# Autodesk Inventor assembly: 3段目
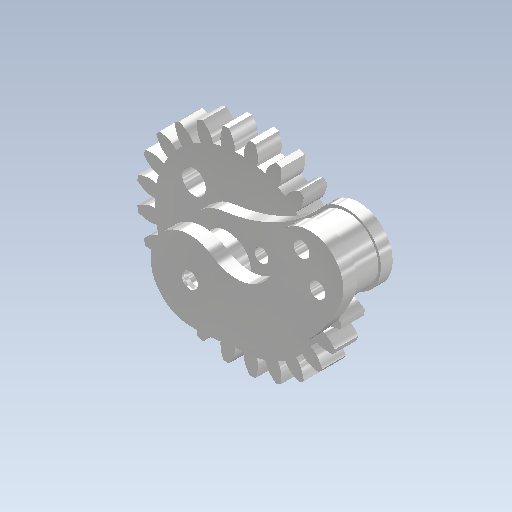
[picture p0: Inventor's stored thumbnail of the model, 512x512]
Saved by Autodesk Inventor 2020.4 (Build 244396000, 396)
## iProperties
Created: 2021-05-01
Part Number: 3段目
Document SubType Name: Assembly
Designer: happy
Mass: 47.1222 g
Surface Area: 125.069 cm^2
Volume: 16.8294 cm^3
Density: 2.8 g/cm^3
Author: happy
## Documents named in this file (9)
- C:\Users\happy\OneDrive\ドキュメント\賢一ファイル\SRDC\試作10-2\アームギア\3段目.iam
- C:\Users\happy\OneDrive\ドキュメント\賢一ファイル\SRDC\試作10-2\アームギア\m2z24.ipt
- C:\Users\happy\OneDrive\ドキュメント\賢一ファイル\SRDC\試作10-2\アームクランク\原動節.ipt
- C:\Users\happy\OneDrive\ドキュメント\賢一ファイル\SRDC\試作10-2\アームギア\3ギア接続部.ipt
- C:\Users\happy\OneDrive\ドキュメント\賢一ファイル\SRDC\試作10-2\アームギア\3ギア接続部外.ipt
- C:\Users\happy\OneDrive\ドキュメント\賢一ファイル\SRDC\試作10-2\アームクランク\原動節2.ipt
- C:\Users\happy\OneDrive\ドキュメント\賢一ファイル\SRDC\試作10-2\アームギア\3ギア接続部2.ipt
- C:\Users\happy\OneDrive\ドキュメント\賢一ファイル\SRDC\試作10-2\アームギア\3ギア接続部3.ipt
- C:\Users\happy\OneDrive\ドキュメント\賢一ファイル\SRDC\試作10-2\アームクランク\原動節つなぎ.ipt
## Components (9 placed, 8 different names)
1. m2z24:1 — 挿入:1, 挿入:2, メイト:1, 挿入:3
2. 原動節:1 — 挿入:1, 挿入:2, 挿入:4, 挿入:9, 挿入:10
3. 3ギア接続部:1 — メイト:1, 挿入:3, メイト:2, 挿入:6
4. 3ギア接続部外:1 — メイト:2, 挿入:4, メイト:3, 挿入:5
5. 3ギア接続部外:2 — メイト:3, 挿入:5, メイト:4, メイト:5, 挿入:8
6. 原動節2:1 — 挿入:8, 挿入:11
7. 3ギア接続部2:1 — メイト:4, 挿入:6, 挿入:7
8. 3ギア接続部3:1 — メイト:5, 挿入:7
9. 原動節つなぎ:1 — 挿入:9, 挿入:10, 挿入:11
## Relationships (16: Insert 11, Mate 5)
- 挿入:1 [Insert]: m2z24:1 ↔ 原動節:1
- 挿入:2 [Insert]: m2z24:1 ↔ 原動節:1
- メイト:1 [Mate]: m2z24:1 ↔ 3ギア接続部:1
- 挿入:3 [Insert]: m2z24:1 ↔ 3ギア接続部:1
- メイト:2 [Mate]: 3ギア接続部:1 ↔ 3ギア接続部外:1
- 挿入:4 [Insert]: 原動節:1 ↔ 3ギア接続部外:1
- メイト:3 [Mate]: 3ギア接続部外:1 ↔ 3ギア接続部外:2
- 挿入:5 [Insert]: 3ギア接続部外:1 ↔ 3ギア接続部外:2
- メイト:4 [Mate]: 3ギア接続部外:2 ↔ 3ギア接続部2:1
- 挿入:6 [Insert]: 3ギア接続部:1 ↔ 3ギア接続部2:1
- メイト:5 [Mate]: 3ギア接続部外:2 ↔ 3ギア接続部3:1
- 挿入:7 [Insert]: 3ギア接続部2:1 ↔ 3ギア接続部3:1
- 挿入:8 [Insert]: 3ギア接続部外:2 ↔ 原動節2:1
- 挿入:9 [Insert]: 原動節:1 ↔ 原動節つなぎ:1
- 挿入:10 [Insert]: 原動節:1 ↔ 原動節つなぎ:1
- 挿入:11 [Insert]: 原動節2:1 ↔ 原動節つなぎ:1
